# Autodesk Inventor assembly: Controls GUI
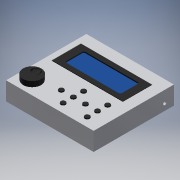
[picture p0: Inventor's stored thumbnail of the model, 180x180]
Saved by Autodesk Inventor 2018 (Build 220112000, 112)
## iProperties
Created: 2017-09-20
Part Number: Controls GUI
Document SubType Name: Assembly
Designer: Gabriel Smolnycki
Author: Gabriel Smolnycki
## Documents named in this file (8)
- E:\planb\mechanics\Subassemblies\Controls GUI assy.iam
- E:\planb\mechanics\Controls\GUI Face.ipt
- E:\planb\mechanics\Controls\GUI Button.ipt
- E:\planb\mechanics\Electronics\4x20 LCD.ipt
- E:\planb\mechanics\Electronics\Keypad.ipt
- E:\planb\mechanics\Controls\GUI Rotary.ipt
- E:\planb\mechanics\Hardware\M3 SS Washer.ipt
- E:\planb\mechanics\Hardware\M3x8 SS SHCS.ipt
## Components (28 placed, 7 different names)
1. GUI Face:1 — Insert:1, Insert:2, Insert:3, Insert:4, Insert:5, Insert:6, Insert:7, Insert:8, Insert:9, Insert:10, Insert:11, Insert:12
2. GUI Button:1 — Insert:8
3. GUI Button:2 — Insert:7
4. GUI Button:3 — Insert:6
5. GUI Button:4 — Insert:5
6. GUI Button:5 — Insert:4
7. GUI Button:6 — Insert:3
8. GUI Button:7 — Insert:2
9. GUI Button:8 — Insert:1
10. 4x20 LCD:1 — Insert:11, Insert:12, Insert:17, Insert:18, Insert:19, Insert:20
11. Keypad:1 — Insert:9, Insert:10, Tangent:1, Mate:1, Mate:2, Insert:13, Insert:14, Insert:15, Insert:16
12. GUI Rotary:1 — Tangent:1, Mate:1, Mate:2
13. M3 SS Washer:1 — Insert:20
14. M3 SS Washer:2 — Insert:19
15. M3 SS Washer:3 — Insert:18
16. M3 SS Washer:4 — Insert:17
17. M3 SS Washer:5 — Insert:16
18. M3 SS Washer:6 — Insert:15
19. M3 SS Washer:7 — Insert:14
20. M3 SS Washer:8 — Insert:13
21. M3x8 SS SHCS:1
22. M3x8 SS SHCS:2
23. M3x8 SS SHCS:3
24. M3x8 SS SHCS:4
25. M3x8 SS SHCS:5
26. M3x8 SS SHCS:6
27. M3x8 SS SHCS:7
28. M3x8 SS SHCS:8
## Relationships (31: Insert 28, Mate 2, Tangent 1)
- Insert:1: GUI Face:1 ↔ GUI Button:8
- Insert:2: GUI Face:1 ↔ GUI Button:7
- Insert:3: GUI Face:1 ↔ GUI Button:6
- Insert:4: GUI Face:1 ↔ GUI Button:5
- Insert:5: GUI Face:1 ↔ GUI Button:4
- Insert:6: GUI Face:1 ↔ GUI Button:3
- Insert:7: GUI Face:1 ↔ GUI Button:2
- Insert:8: GUI Face:1 ↔ GUI Button:1
- Insert:9: GUI Face:1 ↔ Keypad:1
- Insert:10: GUI Face:1 ↔ Keypad:1
- Insert:11: GUI Face:1 ↔ 4x20 LCD:1
- Insert:12: GUI Face:1 ↔ 4x20 LCD:1
- Tangent:1: Keypad:1 ↔ GUI Rotary:1
- Mate:1 (0.254 mm): Keypad:1 ↔ GUI Rotary:1
- Mate:2: Keypad:1 ↔ GUI Rotary:1
- Insert:13: Keypad:1 ↔ M3 SS Washer:8
- Insert:14: Keypad:1 ↔ M3 SS Washer:7
- Insert:15: Keypad:1 ↔ M3 SS Washer:6
- Insert:16: Keypad:1 ↔ M3 SS Washer:5
- Insert:17: 4x20 LCD:1 ↔ M3 SS Washer:4
- Insert:18: 4x20 LCD:1 ↔ M3 SS Washer:3
- Insert:19: 4x20 LCD:1 ↔ M3 SS Washer:2
- Insert:20: 4x20 LCD:1 ↔ M3 SS Washer:1
- [Insert]: M3 SS Washer:1 ↔ M3x8 SS SHCS:8
- [Insert]: M3 SS Washer:2 ↔ M3x8 SS SHCS:7
- [Insert]: M3 SS Washer:3 ↔ M3x8 SS SHCS:6
- [Insert]: M3 SS Washer:4 ↔ M3x8 SS SHCS:5
- [Insert]: M3 SS Washer:7 ↔ M3x8 SS SHCS:4
- [Insert]: M3 SS Washer:5 ↔ M3x8 SS SHCS:3
- [Insert]: M3 SS Washer:8 ↔ M3x8 SS SHCS:2
- [Insert]: M3 SS Washer:6 ↔ M3x8 SS SHCS:1
